# Autodesk Inventor assembly: R07-100-RNEA
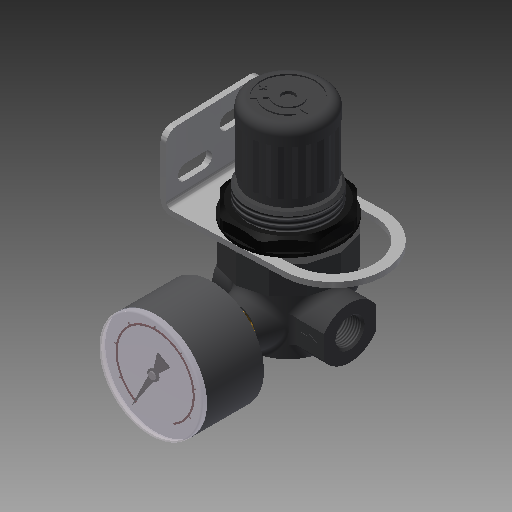
[picture p0: Inventor's stored thumbnail of the model, 512x512]
Saved by Autodesk Inventor 2017 (Build 210142000, 142)
## iProperties
Category: Pneumatics
Company: Autodesk Inc.
Created: 2015-12-11
Part Number: R07-100-RNEA
Document SubType Name: Assembly
Designer: Autodesk Inc.
Catalog Web Link: http://store.norgren.com/us/en/search.aspx?q=r07-100-rnea
Vendor: Norgren
Description: Main Regulator (assembled)
Mass: 112.316 g
Surface Area: 280.109 cm^2
Volume: 88.1678 cm^3
Density: 1.27389 g/cm^3
Author: Autodesk Inc.
## Documents named in this file (5)
- C:\Users\Thariq\Documents\GitHub\bps-bunnybots2016-cad\bps-bunnybots2016-cad\Bunnybot-Night_Fury\15102898-16-A-0000\Pneumatics\Pneu_Norgren_R07-100-RNEA.iam
- C:\Users\Thariq\Documents\GitHub\bps-bunnybots2016-cad\bps-bunnybots2016-cad\Bunnybot-Night_Fury\15102898-16-A-0000\Pneumatics\parts\Pneumatics_Norgren_R07-100-RNEA.ipt
- C:\Users\Thariq\Documents\GitHub\bps-bunnybots2016-cad\bps-bunnybots2016-cad\Bunnybot-Night_Fury\15102898-16-A-0000\Pneumatics\parts\Pneumatics_Norgren_18-025-003_Bracket.ipt
- C:\Users\Thariq\Documents\GitHub\bps-bunnybots2016-cad\bps-bunnybots2016-cad\Bunnybot-Night_Fury\15102898-16-A-0000\Pneumatics\parts\Pneumatics_Norgren_18-025-003_Panel Nut.ipt
- C:\Users\Thariq\Documents\GitHub\bps-bunnybots2016-cad\bps-bunnybots2016-cad\Bunnybot-Night_Fury\15102898-16-A-0000\Pneumatics\Pneu_Norgren_18-013-212.iam
## Components (4 placed, 4 different names)
1. Pneumatics_Norgren_R07-100-RNEA:1 — Mate:1, Mate:2, Mate:3, Insert:1
2. Pneumatics_Norgren_18-025-003_Bracket:1 — Mate:1, Mate:2, Mate:4
3. Pneumatics_Norgren_18-025-003_Panel Nut:1 — Mate:3, Mate:4
4. Pneu_Norgren_18-013-212:1 [sub-assembly] — Insert:1
## Relationships (5: Mate 4, Insert 1)
- Mate:1: Pneumatics_Norgren_R07-100-RNEA:1 ↔ Pneumatics_Norgren_18-025-003_Bracket:1
- Mate:2: Pneumatics_Norgren_R07-100-RNEA:1 ↔ Pneumatics_Norgren_18-025-003_Bracket:1
- Mate:3: Pneumatics_Norgren_R07-100-RNEA:1 ↔ Pneumatics_Norgren_18-025-003_Panel Nut:1
- Mate:4: Pneumatics_Norgren_18-025-003_Bracket:1 ↔ Pneumatics_Norgren_18-025-003_Panel Nut:1
- Insert:1: Pneumatics_Norgren_R07-100-RNEA:1 ↔ Pneu_Norgren_18-013-212:1
